# Autodesk Inventor assembly: Glueholder assembly
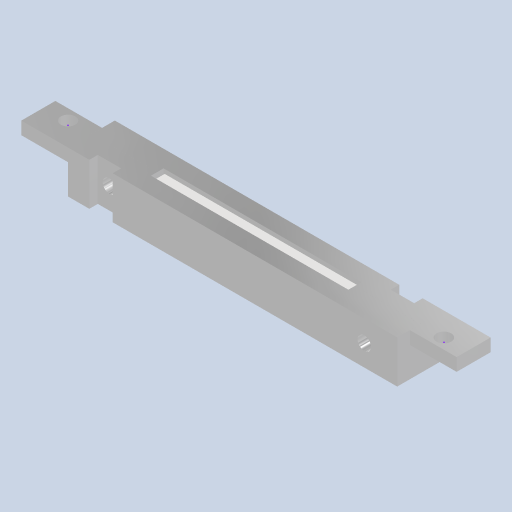
[picture p0: Inventor's stored thumbnail of the model, 512x512]
Saved by Autodesk Inventor 2023.4 (Build 274418000, 418)
## iProperties
Created: 2023-10-31
Part Number: Glueholder assembly
Document SubType Name: Assembly
Designer: PalumaCAD
Author: PalumaCAD
## Documents named in this file (3)
- C:\Users\PalumaCMM\Downloads\Glueholder assembly.iam
- C:\Users\PalumaCMM\Downloads\Glue holder middle block.ipt
- C:\Users\PalumaCMM\Downloads\glue holder.ipt
## Components (3 placed, 2 different names)
1. Glue holder middle block:1 — Mate:3, Mate:4, Flush:2
2. glue holder:1 — Flush:1, Mate:1, Mate:2, Mate:3, Mate:4
3. glue holder:2 — Flush:1, Mate:1, Mate:2, Flush:2
## Relationships (6: Mate 4, Flush 2)
- Flush:1: glue holder:1 ↔ glue holder:2
- Mate:1: glue holder:1 ↔ glue holder:2
- Mate:2: glue holder:1 ↔ glue holder:2
- Mate:3 (0.5 mm): Glue holder middle block:1 ↔ glue holder:1
- Mate:4 (0.25 mm): Glue holder middle block:1 ↔ glue holder:1
- Flush:2 (1 mm): Glue holder middle block:1 ↔ glue holder:2
